# Autodesk Inventor assembly: svejselære
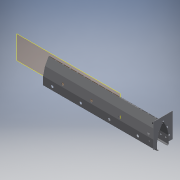
[picture p0: Inventor's stored thumbnail of the model, 180x180]
Saved by Autodesk Inventor 2018 (Build 220112000, 112)
## iProperties
Created: 2019-10-09
Part Number: svejselære
Document SubType Name: Assembly
Designer: loppen
Author: loppen
## Documents named in this file (5)
- H:\INVENTOR 2018\WF_navn_2018\DESIGNS\H4\trappe\svejselære\svejselære.iam
- H:\INVENTOR 2018\WF_navn_2018\DESIGNS\H4\trappe\vange.ipt
- H:\INVENTOR 2018\WF_navn_2018\DESIGNS\H4\trappe\svejselære\svejselære 1.ipt
- H:\INVENTOR 2018\WF_navn_2018\DESIGNS\H4\trappe\svejselære\svejselære 2 del 1.ipt
- H:\INVENTOR 2018\WF_navn_2018\DESIGNS\H4\trappe\svejselære\svejselære 2 del 2.ipt
## Components (4 placed, 4 different names)
1. vange:1 — Flush:1, Flush:2, Flush:6, Flush:7
2. svejselære 1:1 — Flush:1, Flush:2, Flush:3
3. svejselære 2 del 1:1 — Flush:4, Flush:5, Flush:6, Flush:7, Mate:1, Tangent:1, Tangent:2, Mate:2
4. svejselære 2 del 2:1 — Mate:1, Tangent:1, Tangent:2, Mate:2
## Relationships (11: Flush 7, Mate 2, Tangent 2)
- Flush:1: vange:1 ↔ svejselære 1:1
- Flush:2: vange:1 ↔ svejselære 1:1
- Flush:3 (-250 mm): svejselære 1:1
- Flush:4: svejselære 2 del 1:1
- Flush:5: svejselære 2 del 1:1
- Flush:6: vange:1 ↔ svejselære 2 del 1:1
- Flush:7: vange:1 ↔ svejselære 2 del 1:1
- Mate:1: svejselære 2 del 1:1 ↔ svejselære 2 del 2:1
- Tangent:1: svejselære 2 del 1:1 ↔ svejselære 2 del 2:1
- Tangent:2: svejselære 2 del 1:1 ↔ svejselære 2 del 2:1
- Mate:2: svejselære 2 del 1:1 ↔ svejselære 2 del 2:1
